# Autodesk Inventor assembly: A2017_T5_01
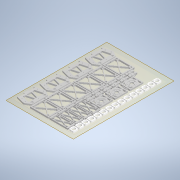
[picture p0: Inventor's stored thumbnail of the model, 180x180]
Saved by Autodesk Inventor 2020 (Build 240168000, 168)
## iProperties
Created: 2021-08-27
Part Number: A2017_T5_01
Document SubType Name: Assembly
Designer: Masato
Author: Masato
## Documents named in this file (8)
- C:\Users\L20C1118 森　圭汰\Documents\2022_0321_open\SUSTAINA-OP\Cam\A2017_T5_01.iam
- C:\Users\L20C1118 森　圭汰\Documents\2022_0321_open\SUSTAINA-OP\Cam\DisposableBoard.ipt
- C:\Users\L20C1118 森　圭汰\Documents\2022_0321_open\SUSTAINA-OP\LowerBody\Knee\Knee_clamp.ipt
- C:\Users\L20C1118 森　圭汰\Documents\2022_0321_open\SUSTAINA-OP\LowerBody\Foot\Foot_root_block.ipt
- C:\Users\L20C1118 森　圭汰\Documents\2022_0321_open\SUSTAINA-OP\UpperBody\Trunk\Trunk_lower_side_frame.ipt
- C:\Users\L20C1118 森　圭汰\Documents\2022_0321_open\SUSTAINA-OP\UpperBody\Arm\Shoulder_horn_frame.ipt
- C:\Users\L20C1118 森　圭汰\Documents\2022_0321_open\SUSTAINA-OP\LowerBody\Link\FrontLink_diagonal.ipt
- C:\Users\L20C1118 森　圭汰\Documents\2022_0321_open\SUSTAINA-OP\LowerBody\Link\BackLink_diagonal.ipt
## Components (45 placed, 7 different names)
1. DisposableBoard:1 — メイト:2, メイト:1, フラッシュ:1, フラッシュ:2, メイト:4, メイト:5, メイト:6, メイト:7, メイト:9, フラッシュ:4, フラッシュ:7, 正接:1, 角度:1, フラッシュ:8, 正接:2, メイト:13
2. FrontLink_diagonal:1 — メイト:6, フラッシュ:4, メイト:10, メイト:12
3. FrontLink_diagonal:2
4. FrontLink_diagonal:3 — メイト:15
5. FrontLink_diagonal:4
6. FrontLink_diagonal:5
7. FrontLink_diagonal:6
8. BackLink_diagonal:1 — メイト:5, メイト:10, フラッシュ:7, 正接:3
9. BackLink_diagonal:2
10. BackLink_diagonal:3
11. BackLink_diagonal:4 — メイト:14, メイト:16
12. Trunk_lower_side_frame:1 — メイト:4, メイト:12, 正接:1, フラッシュ:8
13. Trunk_lower_side_frame:2
14. Trunk_lower_side_frame:3
15. Trunk_lower_side_frame:4
16. Foot_root_block:1 — メイト:9, メイト:15, メイト:16
17. Foot_root_block:2
18. Foot_root_block:3
19. Foot_root_block:4
20. Foot_root_block:5
21. Foot_root_block:6
22. Foot_root_block:7 — メイト:17
23. Foot_root_block:8
24. Foot_root_block:9
25. Foot_root_block:10
26. Foot_root_block:11
27. Foot_root_block:12
28. Knee_clamp:1 — メイト:7, 角度:1, 正接:2, 正接:3
29. Knee_clamp:2
30. Knee_clamp:3
31. Knee_clamp:4
32. Knee_clamp:5
33. Knee_clamp:6
34. Knee_clamp:7
35. Knee_clamp:8
36. Knee_clamp:9
37. Knee_clamp:10
38. Knee_clamp:11
39. Knee_clamp:12
40. Knee_clamp:13
41. Knee_clamp:14
42. Knee_clamp:15
43. Shoulder_horn_frame:2 — メイト:13, メイト:14, メイト:17
44. Shoulder_horn_frame:3
45. Shoulder_horn_frame:4
## Component patterns: (6 elements, first: FrontLink_diagonal:1), (4 elements, first: BackLink_diagonal:1), (4 elements, first: Trunk_lower_side_frame:1), (12 elements, first: Foot_root_block:1), (15 elements, first: Knee_clamp:1), (3 elements, first: Shoulder_horn_frame:2)
## Relationships (23: Mate 14, Flush 5, Tangent 3, Angle 1)
- メイト:2 [Mate]: DisposableBoard:1
- メイト:1 [Mate]: DisposableBoard:1
- フラッシュ:1 [Flush]: DisposableBoard:1
- フラッシュ:2 [Flush]: DisposableBoard:1
- メイト:4 [Mate]: DisposableBoard:1 ↔ Trunk_lower_side_frame:1
- メイト:5 [Mate]: DisposableBoard:1 ↔ BackLink_diagonal:1
- メイト:6 [Mate]: DisposableBoard:1 ↔ FrontLink_diagonal:1
- メイト:7 [Mate]: DisposableBoard:1 ↔ Knee_clamp:1
- メイト:9 [Mate]: DisposableBoard:1 ↔ Foot_root_block:1
- フラッシュ:4 [Flush] (2 mm): DisposableBoard:1 ↔ FrontLink_diagonal:1
- メイト:10 [Mate] (2.5 mm): FrontLink_diagonal:1 ↔ BackLink_diagonal:1
- フラッシュ:7 [Flush] (2 mm): DisposableBoard:1 ↔ BackLink_diagonal:1
- メイト:12 [Mate] (2.5 mm): FrontLink_diagonal:1 ↔ Trunk_lower_side_frame:1
- 正接:1 [Tangent] (2 mm): DisposableBoard:1 ↔ Trunk_lower_side_frame:1
- 角度:1 [Angle] (45 deg): DisposableBoard:1 ↔ Knee_clamp:1
- フラッシュ:8 [Flush] (2 mm): DisposableBoard:1 ↔ Trunk_lower_side_frame:1
- 正接:2 [Tangent] (2 mm): DisposableBoard:1 ↔ Knee_clamp:1
- 正接:3 [Tangent] (2.5 mm): BackLink_diagonal:1 ↔ Knee_clamp:1
- メイト:13 [Mate]: DisposableBoard:1 ↔ Shoulder_horn_frame:2
- メイト:14 [Mate] (2.5 mm): BackLink_diagonal:4 ↔ Shoulder_horn_frame:2
- メイト:15 [Mate] (2.5 mm): FrontLink_diagonal:3 ↔ Foot_root_block:1
- メイト:16 [Mate] (2.5 mm): BackLink_diagonal:4 ↔ Foot_root_block:1
- メイト:17 [Mate] (2.5 mm): Foot_root_block:7 ↔ Shoulder_horn_frame:2
